# Autodesk Inventor assembly: Ground
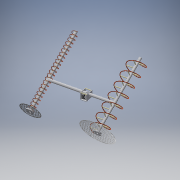
[picture p0: Inventor's stored thumbnail of the model, 180x180]
Saved by Autodesk Inventor 2018 (Build 220112000, 112)
## iProperties
Created: 2018-09-26
Part Number: Ground
Document SubType Name: Assembly
Designer: Bradley
Author: Bradley
## Documents named in this file (4)
- C:\Users\Bradley\Documents\GitHub\CougSat1-Hardware\CougSat1-GroundStation\CADModel\Native\Ground.iam
- C:\Users\Bradley\Documents\GitHub\CougSat1-Hardware\CougSat1-GroundStation\CADModel\Native\Ground_Antenna230mm.iam
- C:\Users\Bradley\Documents\GitHub\CougSat1-Hardware\CougSat1-GroundStation\CADModel\Native\Ground_Antenna700mm.iam
- C:\Users\Bradley\Documents\GitHub\CougSat1-Hardware\CougSat1-GroundStation\CADModel\Native\Ground_Tracker.iam
## Components (3 placed, 3 different names)
1. Ground_Antenna230mm:1 [sub-assembly] — Flush:1, Insert:1
2. Ground_Antenna700mm:1 [sub-assembly] — Insert:2, Mate:1
3. Ground_Tracker:1 [sub-assembly] — Flush:1, Insert:1, Insert:2, Mate:1
## Relationships (4: Insert 2, Flush 1, Mate 1)
- Flush:1: Ground_Antenna230mm:1 ↔ Ground_Tracker:1
- Insert:1: Ground_Antenna230mm:1 ↔ Ground_Tracker:1
- Insert:2: Ground_Antenna700mm:1 ↔ Ground_Tracker:1
- Mate:1: Ground_Antenna700mm:1 ↔ Ground_Tracker:1
